# Autodesk Inventor assembly: 1x1 Male Header 90'
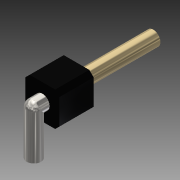
[picture p0: Inventor's stored thumbnail of the model, 180x180]
Saved by Autodesk Inventor 2015 (Build 190159000, 159)
## iProperties
Created: 2016-01-20
Part Number: 1x1 Male Header 90'
Document SubType Name: Assembly
Designer: Kyle
Author: Kyle
## Documents named in this file (4)
- C:\Users\Kyle\Documents\Autodesk\Output\Inventor 2015\Electronics\Headers\Male\1x1 Male Header 90'.iam
- C:\Users\Kyle\Documents\Autodesk\Output\Inventor 2015\Electronics\Sub-Components\Single Bodies\Male Header Base.ipt
- C:\Users\Kyle\Documents\Autodesk\Output\Inventor 2015\Electronics\Sub-Components\Leads\Male Header Lead 90' Straight.ipt
- C:\Users\Kyle\Documents\Autodesk\Output\Inventor 2015\Electronics\Sub-Components\Leads\Male Header Lead 90' Bent.ipt
## Components (3 placed, 3 different names)
1. Male Header Base:1 — Mate:1, Flush:1, Angle:1
2. Male Header Lead 90' Straight:1 — Mate:1, Flush:1, Mate:2, Mate:3
3. Male Header Lead 90' Bent:1 — Mate:2, Mate:3, Angle:1
## Relationships (5: Mate 3, Flush 1, Angle 1)
- Mate:1: Male Header Base:1 ↔ Male Header Lead 90' Straight:1
- Flush:1: Male Header Base:1 ↔ Male Header Lead 90' Straight:1
- Mate:2: Male Header Lead 90' Straight:1 ↔ Male Header Lead 90' Bent:1
- Mate:3: Male Header Lead 90' Straight:1 ↔ Male Header Lead 90' Bent:1
- Angle:1 (0 deg): Male Header Base:1 ↔ Male Header Lead 90' Bent:1
